# Autodesk Inventor assembly: PH50_and_carriage
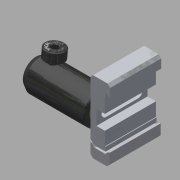
[picture p0: Inventor's stored thumbnail of the model, 180x180]
Saved by Autodesk Inventor 2018 (Build 220112000, 112)
## iProperties
Created: 2018-09-24
Part Number: PH50_and_carriage
Document SubType Name: Assembly
Designer: Robert Campbell
Author: Robert Campbell
## Documents named in this file (3)
- X:\home\work\Documents\MF_BenchOptics\CAD_files\PH50_and_carriage.iam
- X:\home\work\Documents\MF_BenchOptics\CAD_files\PH50_M-Solidworks.ipt
- X:\home\work\Documents\MF_BenchOptics\CAD_files\XT66C4-Step.ipt
## Components (2 placed, 2 different names)
1. PH50_M-Solidworks:1 — Mate:5
2. XT66C4-Step:1 — Mate:5
## Relationships (1: Mate 1)
- Mate:5: PH50_M-Solidworks:1 ↔ XT66C4-Step:1
